# Autodesk Inventor assembly: Planet_Carrier_Modifed_with_sun_gear
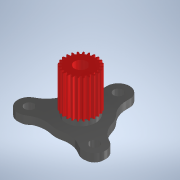
[picture p0: Inventor's stored thumbnail of the model, 180x180]
Saved by Autodesk Inventor 2022 (Build 260153000, 153)
## iProperties
Created: 2022-01-23
Part Number: Planet_Carrier_Modifed_with_sun_gear
Document SubType Name: Assembly
Designer: Mlees
Author: Mlees
## Documents named in this file (3)
- C:\Users\Mlees\Desktop\504Engineering\Stepper-Servo_Based_Robotic_Arm\Designs\Version_4\Created_Parts\Planet_Carrier_Modifed_with_sun_gear.iam
- C:\Users\Mlees\Desktop\504Engineering\Stepper-Servo_Based_Robotic_Arm\Designs\Version_4\Created_Parts\Plamet_Carrier.ipt
- C:\Users\Mlees\Desktop\504Engineering\Stepper-Servo_Based_Robotic_Arm\Designs\Version_4\Created_Parts\24_Teeth_Sun_Gear.ipt
## Components (2 placed, 2 different names)
1. Plamet_Carrier:1 — Rigid:1
2. 24_Teeth_Sun_Gear:1 — Rigid:1
## Relationships (1: WeldJoint 1)
- Rigid:1 [WeldJoint]: Plamet_Carrier:1 ↔ 24_Teeth_Sun_Gear:1
